# Autodesk Inventor assembly: KB33-046-001 - Ходовая часть
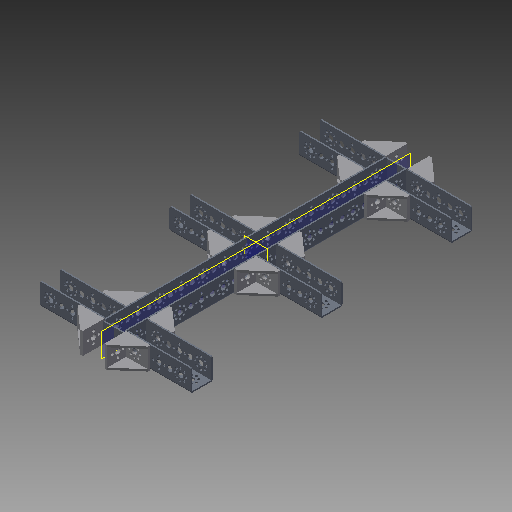
[picture p0: Inventor's stored thumbnail of the model, 512x512]
Saved by Autodesk Inventor 2019 (Build 230136000, 136)
## iProperties
Created: 2021-06-08
Part Number: KB33-046-001 - Ходовая часть
Material: Типовые
Document SubType Name: Assembly
Designer: Петров Иван
Author: Петров Иван
## Documents named in this file (6)
- E:\IVAN\Ivan_desktop\Kvantorium\Projects\RoboPatrol\design\KB33-046-002 - Рама.iam
- E:\IVAN\Ivan_desktop\Kvantorium\Projects\RoboPatrol\design\KB33-046-001-001 - Основание.ipt
- E:\IVAN\Ivan_desktop\Kvantorium\Projects\RoboPatrol\design\standart_components\Tetrix\ftc-tetrix-kit-of-parts-1.snapshot.34\MAX Channels\416mm Channel.ipt
- E:\IVAN\Ivan_desktop\Kvantorium\Projects\RoboPatrol\design\standart_components\Tetrix\ftc-tetrix-kit-of-parts-1.snapshot.34\MAX Channels\96mm Channel.ipt
- E:\IVAN\Ivan_desktop\Kvantorium\Projects\RoboPatrol\design\KB33-046-001-002 - Уголок.ipt
- E:\IVAN\Ivan_desktop\Kvantorium\Projects\RoboPatrol\design\standart_components\Tetrix\ftc-tetrix-kit-of-parts-1.snapshot.34\Brackets\MAX Flat Bracket.ipt
## Components (22 placed, 5 different names)
1. KB33-046-001-001 - Основание:1
2. 416mm Channel:1 — Mate:1, Mate:2, Mate:3, Mate:4, Flush:1, Flush:2, Mate:5, Mate:6, Mate:7
3. MAX Flat Bracket:1 — Mate:11, Mate:12, Mate:13
4. MAX Flat Bracket:2 — Mate:14, Mate:15, Mate:16
5. 96mm Channel:1 — Mate:4, Flush:1, Flush:2, Mate:8, Mate:9, Mate:10, Mate:12
6. KB33-046-001-002 - Уголок:2 — Mate:8, Mate:9, Mate:10
7. KB33-046-001-002 - Уголок:1 — Mate:5, Mate:6, Mate:7
8. 96mm Channel:2
9. KB33-046-001-002 - Уголок:3
10. KB33-046-001-002 - Уголок:5
11. 96mm Channel:3 — Mate:14, Mate:15
12. KB33-046-001-002 - Уголок:4
13. KB33-046-001-002 - Уголок:6
14. 96mm Channel:4 — Mate:16
15. KB33-046-001-002 - Уголок:7
16. KB33-046-001-002 - Уголок:8
17. 96mm Channel:5
18. KB33-046-001-002 - Уголок:9
19. KB33-046-001-002 - Уголок:10
20. 96mm Channel:6 — Mate:11, Mate:13
21. KB33-046-001-002 - Уголок:11
22. KB33-046-001-002 - Уголок:12
## Component patterns: (2 elements), (3 elements, first: 96mm Channel:1 + KB33-046-001-002 - Уголок:2 + KB33-046-001-002 - Уголок:1), Component Pattern 1:2 (3 elements)
## Relationships (18: Mate 16, Flush 2)
- Mate:1: 416mm Channel:1
- Mate:2: 416mm Channel:1
- Mate:3: 416mm Channel:1
- Mate:4: 416mm Channel:1 ↔ 96mm Channel:1
- Flush:1: 416mm Channel:1 ↔ 96mm Channel:1
- Flush:2: 416mm Channel:1 ↔ 96mm Channel:1
- Mate:5: 416mm Channel:1 ↔ KB33-046-001-002 - Уголок:1
- Mate:6: 416mm Channel:1 ↔ KB33-046-001-002 - Уголок:1
- Mate:7: 416mm Channel:1 ↔ KB33-046-001-002 - Уголок:1
- Mate:8: 96mm Channel:1 ↔ KB33-046-001-002 - Уголок:2
- Mate:9: 96mm Channel:1 ↔ KB33-046-001-002 - Уголок:2
- Mate:10: 96mm Channel:1 ↔ KB33-046-001-002 - Уголок:2
- Mate:11: MAX Flat Bracket:1 ↔ 96mm Channel:6
- Mate:12: MAX Flat Bracket:1 ↔ 96mm Channel:1
- Mate:13: MAX Flat Bracket:1 ↔ 96mm Channel:6
- Mate:14: MAX Flat Bracket:2 ↔ 96mm Channel:3
- Mate:15: MAX Flat Bracket:2 ↔ 96mm Channel:3
- Mate:16: MAX Flat Bracket:2 ↔ 96mm Channel:4
